# Autodesk Inventor assembly: EnsambleTuberiaPaso
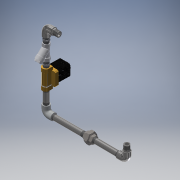
[picture p0: Inventor's stored thumbnail of the model, 180x180]
Saved by Autodesk Inventor 2017 (Build 210142000, 142)
## iProperties
Created: 2021-06-28
Part Number: EnsambleTuberiaPaso
Document SubType Name: Assembly
Designer: USUARIO
Author: USUARIO
## Documents named in this file (10)
- D:\Laboratorio\Autoclave\Autoclave Horizontal\Con Precamara\2021\Autoclave 110L Biocacol OP2021110 #0045886XX\Modelo\Planos\EnsambleTuberiaPaso.iam
- C:\Modelos 3D y DXF\Racores\CodoCalle.iam
- C:\Modelos 3D y DXF\Filtro en Y\Filtro Y 1-2'' Inox.ipt
- C:\Modelos 3D y DXF\Racores\B122 1-2x1-2.ipt
- C:\Modelos 3D y DXF\Danfoss EV210B\DANFOS EV225B.ipt
- C:\Modelos 3D y DXF\Racores\Niple 1-2x3.ipt
- C:\Modelos 3D y DXF\Racores\User Library-codo a 90 de 1-2-Rosc.ipt
- C:\Modelos 3D y DXF\Racores\Universal1-2.ipt
- C:\Modelos 3D y DXF\Racores\Niple 1-2x5.ipt
- C:\Modelos 3D y DXF\Racores\Niple 1-2x6.ipt
## Components (11 placed, 9 different names)
1. CodoCalle:1 [sub-assembly]
2. Filtro Y 1-2'' Inox:1
3. B122 1-2x1-2:1
4. CodoCalle:2 [sub-assembly]
5. B122 1-2x1-2:2
6. DANFOS EV225B:1
7. Niple 1-2x3:1
8. User Library-codo a 90 de 1-2-Rosc:1
9. Universal1-2:1
10. Niple 1-2x5:1
11. Niple 1-2x6:1
## Relationships (9: Insert 9)
- [Insert] (-9 mm): CodoCalle:1 ↔ B122 1-2x1-2:1
- [Insert] (7 mm): Filtro Y 1-2'' Inox:1 ↔ B122 1-2x1-2:1
- [Insert] (-7 mm): Filtro Y 1-2'' Inox:1 ↔ B122 1-2x1-2:2
- [Insert] (-10 mm): B122 1-2x1-2:2 ↔ DANFOS EV225B:1
- [Insert] (-12 mm): DANFOS EV225B:1 ↔ Niple 1-2x3:1
- [Insert] (-10 mm): Niple 1-2x3:1 ↔ User Library-codo a 90 de 1-2-Rosc:1
- [Insert] (-12 mm): CodoCalle:2 ↔ Niple 1-2x5:1
- [Insert] (-12 mm): Universal1-2:1 ↔ Niple 1-2x5:1
- [Insert] (-12 mm): User Library-codo a 90 de 1-2-Rosc:1 ↔ Niple 1-2x6:1
